# Autodesk Inventor assembly: ShootingMechanism
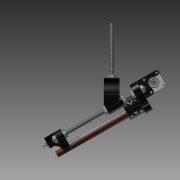
[picture p0: Inventor's stored thumbnail of the model, 180x180]
Saved by Autodesk Inventor 2015 (Build 190159000, 159)
## iProperties
Created: 2017-01-04
Part Number: ShootingMechanism
Document SubType Name: Assembly
Designer: Ernest
Mass: 501.827 g
Surface Area: 1553.31 cm^2
Volume: 501.827 cm^3
Density: 1 g/cm^3
Author: Ernest
## Documents named in this file (20)
- C:\Users\Ernest\Documents\Capstone-Project\doc\CAD\ShootingMechanism\ShootingMechanism.iam
- C:\Users\Ernest\Documents\Capstone-Project\doc\CAD\ShootingMechanism\CueStickTip.ipt
- C:\Users\Ernest\Documents\Capstone-Project\doc\CAD\ShootingMechanism\ThreadedBar.ipt
- C:\Users\Ernest\Documents\Capstone-Project\doc\CAD\ShootingMechanism\SmoothBar.ipt
- C:\Users\Ernest\Documents\Capstone-Project\doc\CAD\ShootingMechanism\ThreadBarNut.ipt
- C:\Users\Ernest\Documents\Capstone-Project\doc\CAD\ShootingMechanism\LinearBearing.ipt
- C:\Users\Ernest\Documents\Capstone-Project\doc\CAD\ShootingMechanism\NEMA 17 with T5 Pulley.iam
- C:\Users\Ernest\Documents\Capstone-Project\doc\CAD\ShootingMechanism\FrontStopper.ipt
- C:\Users\Ernest\Documents\Capstone-Project\doc\CAD\ShootingMechanism\IdlePulley.ipt
- C:\Users\Ernest\Documents\Capstone-Project\doc\CAD\ShootingMechanism\PulleyScrew.ipt
- C:\Users\Ernest\Documents\Capstone-Project\doc\CAD\ShootingMechanism\PulleyHolder.ipt
- C:\Users\Ernest\Documents\Capstone-Project\doc\CAD\ShootingMechanism\PulleyNut.ipt
- C:\Users\Ernest\Documents\Capstone-Project\doc\CAD\ShootingMechanism\BackStopper.ipt
- C:\Users\Ernest\Documents\Capstone-Project\doc\CAD\ShootingMechanism\Spring.ipt
- C:\Users\Ernest\Documents\Capstone-Project\doc\CAD\ShootingMechanism\MountBar.ipt
- C:\Users\Ernest\Documents\Capstone-Project\doc\CAD\ShootingMechanism\MountB.ipt
- C:\Users\Ernest\Documents\Capstone-Project\doc\CAD\ShootingMechanism\CueHolderTop.ipt
- C:\Users\Ernest\Documents\Capstone-Project\doc\CAD\ShootingMechanism\CueHolderLBBottom.ipt
- C:\Users\Ernest\Documents\Capstone-Project\doc\CAD\ShootingMechanism\CueHolderBottom.ipt
- C:\Users\Ernest\Documents\Capstone-Project\doc\CAD\ShootingMechanism\CueBeltHorder.ipt
## Components (62 placed, 19 different names)
1. CueStickTip:1 — Mate:20, Flush:2
2. ThreadedBar:1 — Mate:2, Mate:6, Mate:7, Mate:10, Mate:11, Flush:6, Flush:7, Mate:77, Mate:78, Mate:89
3. ThreadedBar:2 — Mate:3, Mate:4, Mate:5, Mate:8, Mate:9, Flush:6, Mate:75, Mate:76, Mate:90
4. SmoothBar:1 — Mate:12, Flush:3, Mate:21, Mate:40, Mate:42, Mate:95
5. SmoothBar:2 — Mate:13, Flush:3, Mate:41, Mate:96
6. ThreadBarNut:1 — Mate:9, Mate:45
7. ThreadBarNut:2 — Mate:4, Mate:22
8. ThreadBarNut:3 — Mate:11, Mate:44
9. ThreadBarNut:4 — Mate:6, Mate:25
10. ThreadBarNut:5 — Mate:10, Mate:43
11. ThreadBarNut:6 — Mate:7, Mate:23
12. ThreadBarNut:7 — Mate:8, Mate:46
13. ThreadBarNut:8 — Mate:5, Mate:24
14. LinearBearing:1 — Flush:1, Mate:96, Mate:97, Mate:101
15. LinearBearing:2 — Flush:1, Flush:2, Mate:95, Mate:98, Flush:39
16. NEMA 17 with T5 Pulley:1 [sub-assembly] — Angle:1, Angle:2, Flush:8, Mate:47, Mate:48
17. FrontStopper:1 — Mate:2, Mate:3, Mate:12, Mate:13, Mate:20, Mate:21, Mate:22, Mate:23, Mate:24, Mate:25, Mate:35, Mate:36, Mate:37, Mate:38, Mate:39, Angle:3
18. IdlePulley:1 — Mate:26, Mate:33
19. PulleyScrew:1 — Mate:26, Mate:27, Mate:28, Mate:29
20. PulleyHolder:1 — Mate:28, Mate:29, Mate:30, Mate:31, Mate:32, Mate:33, Mate:36
21. PulleyNut:1 — Mate:27, Mate:30
22. PulleyScrew:2 — Mate:31, Mate:32, Mate:34, Mate:35, Flush:4
23. PulleyNut:2 — Mate:34, Flush:4
24. BackStopper:1 — Mate:37, Mate:42, Mate:43, Mate:44, Mate:45, Mate:46, Flush:7, Angle:1, Angle:2, Angle:3, Flush:8, Mate:47, Mate:48, Mate:49, Mate:50, Mate:51, Mate:52
25. Spring:1 — Mate:39, Mate:40
26. Spring:2 — Mate:38, Mate:41
27. PulleyScrew:3 — Mate:49, Flush:10
28. PulleyScrew:4 — Mate:51, Flush:9
29. PulleyScrew:5 — Mate:50, Flush:9, Flush:10, Mate:52
30. MountB:1 — Mate:86, Mate:87, Mate:88, Mate:89, Mate:90, Mate:91, Mate:92
31. ThreadBarNut:15 — Mate:76, Flush:15
32. ThreadBarNut:16 — Mate:75, Flush:16
33. ThreadBarNut:17 — Mate:77, Flush:15, Mate:92
34. ThreadBarNut:18 — Mate:78, Flush:16, Mate:91
35. MountBar:2 — Mate:84, Mate:85, Flush:14, Mate:88
36. ThreadBarNut:19 — Mate:84, Mate:87
37. ThreadBarNut:20 — Mate:85, Flush:14, Mate:86
38. CueHolderLBBottom:1 — Mate:97, Flush:19, Flush:41
39. CueHolderLBBottom:2 — Mate:98, Flush:19, Mate:102, Mate:134, Flush:40
40. CueHolderBottom:1 — Mate:103, Mate:104, Mate:105, Mate:135
41. CueHolderTop:1 — Mate:101, Mate:102, Mate:103, Mate:104, Mate:105, Mate:108, Mate:109, Mate:110, Mate:111, Mate:112, Mate:113, Mate:114, Mate:115, Mate:116, Mate:117, Mate:118, Mate:119, Mate:120, Mate:122, Mate:125, Mate:136, Mate:137, Flush:39, Flush:40, Flush:41
42. CueBeltHorder:1 — Mate:108, Mate:109, Mate:110
43. PulleyScrew:6 — Mate:113, Mate:126, Flush:38
44. PulleyScrew:7 — Mate:116, Flush:22, Mate:131
45. PulleyScrew:8 — Mate:112, Flush:28, Mate:122, Mate:124
46. PulleyScrew:9 — Mate:117, Flush:21, Flush:22, Flush:25, Mate:132
47. PulleyScrew:10 — Mate:115, Flush:21, Mate:130
48. PulleyScrew:11 — Mate:118, Flush:23, Mate:128
49. PulleyScrew:12 — Mate:120, Flush:23, Flush:24, Flush:25, Mate:129, Mate:136
50. PulleyScrew:13 — Mate:119, Flush:24, Mate:127
51. PulleyScrew:14 — Mate:114, Mate:133, Flush:38, Mate:137
52. PulleyScrew:15 — Mate:111, Flush:28, Mate:123
53. PulleyNut:3 — Mate:123, Flush:29, Mate:125
54. PulleyNut:4 — Mate:124, Flush:29
55. PulleyNut:5 — Flush:31, Flush:32, Mate:126, Mate:134
56. PulleyNut:6 — Flush:31, Mate:127
57. PulleyNut:7 — Mate:128, Flush:37
58. PulleyNut:8 — Flush:33, Mate:131
59. PulleyNut:9 — Flush:36, Mate:129, Flush:37, Mate:135
60. PulleyNut:10 — Flush:35, Mate:132
61. PulleyNut:11 — Flush:35, Flush:36, Mate:130
62. PulleyNut:12 — Flush:32, Flush:33, Mate:133
## Relationships (129: Mate 96, Flush 30, Angle 3)
- Mate:2: ThreadedBar:1 ↔ FrontStopper:1
- Mate:3: ThreadedBar:2 ↔ FrontStopper:1
- Mate:4: ThreadedBar:2 ↔ ThreadBarNut:2
- Mate:5: ThreadedBar:2 ↔ ThreadBarNut:8
- Mate:6: ThreadedBar:1 ↔ ThreadBarNut:4
- Mate:7: ThreadedBar:1 ↔ ThreadBarNut:6
- Mate:8: ThreadedBar:2 ↔ ThreadBarNut:7
- Mate:9: ThreadedBar:2 ↔ ThreadBarNut:1
- Mate:10: ThreadedBar:1 ↔ ThreadBarNut:5
- Mate:11: ThreadedBar:1 ↔ ThreadBarNut:3
- Mate:12: SmoothBar:1 ↔ FrontStopper:1
- Mate:13: SmoothBar:2 ↔ FrontStopper:1
- Mate:20: CueStickTip:1 ↔ FrontStopper:1
- Flush:1: LinearBearing:1 ↔ LinearBearing:2
- Flush:2: CueStickTip:1 ↔ LinearBearing:2
- Flush:3: SmoothBar:1 ↔ SmoothBar:2
- Mate:21: SmoothBar:1 ↔ FrontStopper:1
- Mate:22: ThreadBarNut:2 ↔ FrontStopper:1
- Mate:23: ThreadBarNut:6 ↔ FrontStopper:1
- Mate:24: ThreadBarNut:8 ↔ FrontStopper:1
- Mate:25: ThreadBarNut:4 ↔ FrontStopper:1
- Mate:26: IdlePulley:1 ↔ PulleyScrew:1
- Mate:27: PulleyScrew:1 ↔ PulleyNut:1
- Mate:28: PulleyScrew:1 ↔ PulleyHolder:1
- Mate:29: PulleyScrew:1 ↔ PulleyHolder:1
- Mate:30: PulleyHolder:1 ↔ PulleyNut:1
- Mate:31: PulleyHolder:1 ↔ PulleyScrew:2
- Mate:32: PulleyHolder:1 ↔ PulleyScrew:2
- Mate:33 (1.5 mm): IdlePulley:1 ↔ PulleyHolder:1
- Mate:34: PulleyScrew:2 ↔ PulleyNut:2
- Mate:35: FrontStopper:1 ↔ PulleyScrew:2
- Mate:36: FrontStopper:1 ↔ PulleyHolder:1
- Flush:4 (-6.332 mm): PulleyScrew:2 ↔ PulleyNut:2
- Mate:37: FrontStopper:1 ↔ BackStopper:1
- Mate:38: FrontStopper:1 ↔ Spring:2
- Mate:39: FrontStopper:1 ↔ Spring:1
- Mate:40: SmoothBar:1 ↔ Spring:1
- Mate:41: SmoothBar:2 ↔ Spring:2
- Mate:42: SmoothBar:1 ↔ BackStopper:1
- Flush:6: ThreadedBar:1 ↔ ThreadedBar:2
- Mate:43: ThreadBarNut:5 ↔ BackStopper:1
- Mate:44: ThreadBarNut:3 ↔ BackStopper:1
- Mate:45: ThreadBarNut:1 ↔ BackStopper:1
- Mate:46: ThreadBarNut:7 ↔ BackStopper:1
- Flush:7 (-10 mm): ThreadedBar:1 ↔ BackStopper:1
- Angle:1 (90 deg): NEMA 17 with T5 Pulley:1 ↔ BackStopper:1
- Angle:2 (90 deg): NEMA 17 with T5 Pulley:1 ↔ BackStopper:1
- Angle:3 (0 deg): FrontStopper:1 ↔ BackStopper:1
- Flush:8: NEMA 17 with T5 Pulley:1 ↔ BackStopper:1
- Mate:47: NEMA 17 with T5 Pulley:1 ↔ BackStopper:1
- Mate:48: NEMA 17 with T5 Pulley:1 ↔ BackStopper:1
- Mate:49: BackStopper:1 ↔ PulleyScrew:3
- Mate:50: BackStopper:1 ↔ PulleyScrew:5
- Mate:51: BackStopper:1 ↔ PulleyScrew:4
- Flush:9: PulleyScrew:4 ↔ PulleyScrew:5
- Flush:10: PulleyScrew:3 ↔ PulleyScrew:5
- Mate:52: BackStopper:1 ↔ PulleyScrew:5
- Mate:75: ThreadedBar:2 ↔ ThreadBarNut:16
- Mate:76: ThreadedBar:2 ↔ ThreadBarNut:15
- Mate:77: ThreadedBar:1 ↔ ThreadBarNut:17
- Mate:78: ThreadedBar:1 ↔ ThreadBarNut:18
- Mate:84: MountBar:2 ↔ ThreadBarNut:19
- Mate:85: MountBar:2 ↔ ThreadBarNut:20
- Flush:14 (0.2 mm): MountBar:2 ↔ ThreadBarNut:20
- Mate:86: MountB:1 ↔ ThreadBarNut:20
- Mate:87: MountB:1 ↔ ThreadBarNut:19
- Mate:88: MountB:1 ↔ MountBar:2
- Mate:89: ThreadedBar:1 ↔ MountB:1
- Mate:90: ThreadedBar:2 ↔ MountB:1
- Flush:15: ThreadBarNut:15 ↔ ThreadBarNut:17
- Flush:16: ThreadBarNut:16 ↔ ThreadBarNut:18
- Mate:91: MountB:1 ↔ ThreadBarNut:18
- Mate:92: MountB:1 ↔ ThreadBarNut:17
- Mate:95: SmoothBar:1 ↔ LinearBearing:2
- Mate:96: SmoothBar:2 ↔ LinearBearing:1
- Mate:97: LinearBearing:1 ↔ CueHolderLBBottom:1
- Mate:98: LinearBearing:2 ↔ CueHolderLBBottom:2
- Flush:19: CueHolderLBBottom:1 ↔ CueHolderLBBottom:2
- Mate:101: LinearBearing:1 ↔ CueHolderTop:1
- Mate:102: CueHolderLBBottom:2 ↔ CueHolderTop:1
- Mate:103: CueHolderBottom:1 ↔ CueHolderTop:1
- Mate:104: CueHolderBottom:1 ↔ CueHolderTop:1
- Mate:105: CueHolderBottom:1 ↔ CueHolderTop:1
- Mate:108: CueHolderTop:1 ↔ CueBeltHorder:1
- Mate:109: CueHolderTop:1 ↔ CueBeltHorder:1
- Mate:110: CueHolderTop:1 ↔ CueBeltHorder:1
- Mate:111: CueHolderTop:1 ↔ PulleyScrew:15
- Mate:112: CueHolderTop:1 ↔ PulleyScrew:8
- Mate:113: CueHolderTop:1 ↔ PulleyScrew:6
- Mate:114: CueHolderTop:1 ↔ PulleyScrew:14
- Mate:115: CueHolderTop:1 ↔ PulleyScrew:10
- Mate:116: CueHolderTop:1 ↔ PulleyScrew:7
- Mate:117: CueHolderTop:1 ↔ PulleyScrew:9
- Mate:118: CueHolderTop:1 ↔ PulleyScrew:11
- Mate:119: CueHolderTop:1 ↔ PulleyScrew:13
- Mate:120: CueHolderTop:1 ↔ PulleyScrew:12
- Flush:21: PulleyScrew:9 ↔ PulleyScrew:10
- Flush:22: PulleyScrew:7 ↔ PulleyScrew:9
- Flush:23: PulleyScrew:11 ↔ PulleyScrew:12
- Flush:24: PulleyScrew:12 ↔ PulleyScrew:13
- Flush:25: PulleyScrew:9 ↔ PulleyScrew:12
- Flush:28: PulleyScrew:8 ↔ PulleyScrew:15
- Mate:122: CueHolderTop:1 ↔ PulleyScrew:8
- Mate:123: PulleyScrew:15 ↔ PulleyNut:3
- Mate:124: PulleyScrew:8 ↔ PulleyNut:4
- Flush:29: PulleyNut:3 ↔ PulleyNut:4
- Mate:125: CueHolderTop:1 ↔ PulleyNut:3
- Flush:31: PulleyNut:5 ↔ PulleyNut:6
- Flush:32: PulleyNut:5 ↔ PulleyNut:12
- Flush:33: PulleyNut:8 ↔ PulleyNut:12
- Flush:35: PulleyNut:10 ↔ PulleyNut:11
- Flush:36: PulleyNut:9 ↔ PulleyNut:11
- Mate:126: PulleyScrew:6 ↔ PulleyNut:5
- Mate:127: PulleyScrew:13 ↔ PulleyNut:6
- Mate:128: PulleyScrew:11 ↔ PulleyNut:7
- Mate:129: PulleyScrew:12 ↔ PulleyNut:9
- Mate:130: PulleyScrew:10 ↔ PulleyNut:11
- Mate:131: PulleyScrew:7 ↔ PulleyNut:8
- Mate:132: PulleyScrew:9 ↔ PulleyNut:10
- Mate:133: PulleyScrew:14 ↔ PulleyNut:12
- Flush:37: PulleyNut:7 ↔ PulleyNut:9
- Mate:134: CueHolderLBBottom:2 ↔ PulleyNut:5
- Mate:135: CueHolderBottom:1 ↔ PulleyNut:9
- Mate:136: CueHolderTop:1 ↔ PulleyScrew:12
- Flush:38: PulleyScrew:6 ↔ PulleyScrew:14
- Mate:137: CueHolderTop:1 ↔ PulleyScrew:14
- Flush:39: LinearBearing:2 ↔ CueHolderTop:1
- Flush:40: CueHolderLBBottom:2 ↔ CueHolderTop:1
- Flush:41: CueHolderLBBottom:1 ↔ CueHolderTop:1
